# Autodesk Inventor assembly: ENSAMBLE GENERAL ACH-40L-2020-V
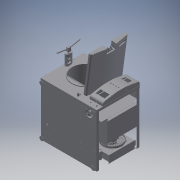
[picture p0: Inventor's stored thumbnail of the model, 180x180]
Saved by Autodesk Inventor 2017 (Build 210142000, 142)
## iProperties
Created: 2020-09-24
Part Number: ENSAMBLE GENERAL ACH-40L-2020-V
Description: STEP AP203
Document SubType Name: Assembly
Designer: USUARIO
Sending System: SolidWorks 2013
Preprocessor: SwSTEP 2.0
Title: ENSAMBLE GENERAL ACH-40L-2020-V.STEP
Revision Number: ANY
## Documents named in this file (46)
- D:\Laboratorio\Autoclave\Autoclave Horizontal\Sin Precamara\2020\Autoclave 40L con Vacio Insulab #0045883XX OP2020292\Ensamble General\ENSAMBLE GENERAL ACH-40L-2020-V.iam
- D:\Laboratorio\Autoclave\Autoclave Horizontal\Sin Precamara\2020\Autoclave 40L con Vacio Insulab #0045883XX OP2020292\Ensamble General\CUBIERTA FRONTAL ACH-40L-2020-V.ipt
- D:\Laboratorio\Autoclave\Autoclave Horizontal\Sin Precamara\2020\Autoclave 40L con Vacio Insulab #0045883XX OP2020292\Ensamble General\BASE MUEBLE ACH-40L-2020-V.ipt
- D:\Laboratorio\Autoclave\Autoclave Horizontal\Sin Precamara\2020\Autoclave 40L con Vacio Insulab #0045883XX OP2020292\Ensamble General\MARCO POSTERIOR ACH-40L-2020-V.ipt
- D:\Laboratorio\Autoclave\Autoclave Horizontal\Sin Precamara\2020\Autoclave 40L con Vacio Insulab #0045883XX OP2020292\Ensamble General\ENSAMBLE TANQUE ACH-40L-2020-V.iam
- D:\Laboratorio\Autoclave\Autoclave Horizontal\Sin Precamara\2020\Autoclave 40L con Vacio Insulab #0045883XX OP2020292\Ensamble General\ENSAMBLE PANEL FRONTAL ACH-40L-2020-V.iam
- D:\Laboratorio\Autoclave\Autoclave Horizontal\Sin Precamara\2020\Autoclave 40L con Vacio Insulab #0045883XX OP2020292\Ensamble General\ENSAMBLE PUERTA ACH-40L-2020-V.iam
- D:\Laboratorio\Autoclave\Autoclave Horizontal\Sin Precamara\2020\Autoclave 40L con Vacio Insulab #0045883XX OP2020292\Ensamble General\CAJA CONEXIONES ESPINAS ACH-40L-2020-V.ipt
- D:\Laboratorio\Autoclave\Autoclave Horizontal\Sin Precamara\2020\Autoclave 40L con Vacio Insulab #0045883XX OP2020292\Ensamble General\PG-13,5.ipt
- D:\Laboratorio\Autoclave\Autoclave Horizontal\Sin Precamara\2020\Autoclave 40L con Vacio Insulab #0045883XX OP2020292\Ensamble General\CAJA CONEXIONES ACH-40L-2020-V.ipt
- D:\Laboratorio\Autoclave\Autoclave Horizontal\Sin Precamara\2020\Autoclave 40L con Vacio Insulab #0045883XX OP2020292\Ensamble General\REFUERZO INTERIOR ACH-40L-2020-V.ipt
- D:\Laboratorio\Autoclave\Autoclave Horizontal\Sin Precamara\2020\Autoclave 40L con Vacio Insulab #0045883XX OP2020292\Ensamble General\VENTILADOR 9X9.ipt
- D:\Laboratorio\Autoclave\Autoclave Horizontal\Sin Precamara\2020\Autoclave 40L con Vacio Insulab #0045883XX OP2020292\Ensamble General\ENSAMBLE GENERAL CIERRE JP2019-TTNR.iam
- D:\Laboratorio\Autoclave\Autoclave Horizontal\Sin Precamara\2020\Autoclave 40L con Vacio Insulab #0045883XX OP2020292\Ensamble General\PIN CIERRE JP2019-TTNR.ipt
- D:\Laboratorio\Autoclave\Autoclave Horizontal\Sin Precamara\2020\Autoclave 40L con Vacio Insulab #0045883XX OP2020292\Ensamble General\PIN BISAGRA JP2019-TTNR.ipt
- D:\Laboratorio\Autoclave\Autoclave Horizontal\Sin Precamara\2020\Autoclave 40L con Vacio Insulab #0045883XX OP2020292\Ensamble General\PIVOTE CIERRE JP2019-TTNR.ipt
- D:\Laboratorio\Autoclave\Autoclave Horizontal\Sin Precamara\2020\Autoclave 40L con Vacio Insulab #0045883XX OP2020292\Ensamble General\ENSAMBLE TAPA ACH-40L-2020-V.iam
- D:\Laboratorio\Autoclave\Autoclave Horizontal\Sin Precamara\2020\Autoclave 40L con Vacio Insulab #0045883XX OP2020292\Ensamble General\ENSAMBLE RESERVORIO ACH-40L-2020-V.iam
- D:\Laboratorio\Autoclave\Autoclave Horizontal\Sin Precamara\2020\Autoclave 40L con Vacio Insulab #0045883XX OP2020292\Ensamble General\CONTRATAPA SUPERIOR ACH-40L-2020-V.ipt
- D:\Laboratorio\Autoclave\Autoclave Horizontal\Sin Precamara\2020\Autoclave 40L con Vacio Insulab #0045883XX OP2020292\Ensamble General\BANDEJA INTERIOR ACH-40L-2020-V.ipt
- D:\Laboratorio\Autoclave\Autoclave Horizontal\Sin Precamara\2020\Autoclave 40L con Vacio Insulab #0045883XX OP2020292\Ensamble General\BOMBA DE VACIO THOMAS 2107CA20.ipt
- D:\Laboratorio\Autoclave\Autoclave Horizontal\Sin Precamara\2020\Autoclave 40L con Vacio Insulab #0045883XX OP2020292\Ensamble General\CALDERIN ACH-40L-2020-V.ipt
- D:\Laboratorio\Autoclave\Autoclave Horizontal\Sin Precamara\2020\Autoclave 40L con Vacio Insulab #0045883XX OP2020292\Ensamble General\CONTRATAPA INFERIOR ACH-40L-2020-V.ipt
- D:\Laboratorio\Autoclave\Autoclave Horizontal\Sin Precamara\2020\Autoclave 40L con Vacio Insulab #0045883XX OP2020292\Ensamble General\CUBIERTA SUPERIOR ACH-40L-2020-V.ipt
- D:\Laboratorio\Autoclave\Autoclave Horizontal\Sin Precamara\2020\Autoclave 40L con Vacio Insulab #0045883XX OP2020292\Ensamble General\CUBIERTA LATERAL ACH-40L-2020-V.ipt
- D:\Laboratorio\Autoclave\Autoclave Horizontal\Sin Precamara\2020\Autoclave 40L con Vacio Insulab #0045883XX OP2020292\Ensamble General\ENSAMBLE RADIADOR ACH-40L-2020-V.iam
- D:\Laboratorio\Autoclave\Autoclave Horizontal\Sin Precamara\2020\Autoclave 40L con Vacio Insulab #0045883XX OP2020292\Ensamble General\CUBIERTA LATERAL DERECHA ACH-40L-2020-V.ipt
- D:\Laboratorio\Autoclave\Autoclave Horizontal\Sin Precamara\2020\Autoclave 40L con Vacio Insulab #0045883XX OP2020292\Ensamble General\CUBIERTA POSTERIOR ACH-40L-2020-V.ipt
- D:\Laboratorio\Autoclave\Autoclave Horizontal\Sin Precamara\2020\Autoclave 40L con Vacio Insulab #0045883XX OP2020292\Ensamble General\ULKA EX5.ipt
- D:\Laboratorio\Autoclave\Autoclave Horizontal\Sin Precamara\2020\Autoclave 40L con Vacio Insulab #0045883XX OP2020292\Ensamble General\DANFOSS EV215B.ipt
- D:\Laboratorio\Autoclave\Autoclave Horizontal\Sin Precamara\2020\Autoclave 40L con Vacio Insulab #0045883XX OP2020292\Ensamble General\SOPORTE BOMBA AGUA ACH-40L-2020-V.ipt
- D:\Laboratorio\Autoclave\Autoclave Horizontal\Sin Precamara\2020\Autoclave 40L con Vacio Insulab #0045883XX OP2020292\Ensamble General\SOPORTE VALVULAS ACH-40L-2020-V.ipt
- D:\Laboratorio\Autoclave\Autoclave Horizontal\Sin Precamara\2020\Autoclave 40L con Vacio Insulab #0045883XX OP2020292\Ensamble General\PATA 5-16.ipt
- D:\Laboratorio\Autoclave\Autoclave Horizontal\Sin Precamara\2020\Autoclave 40L con Vacio Insulab #0045883XX OP2020292\Ensamble General\VALVULA DE BOLA GENEBRE MH 3097-02 CW617N.ipt
- D:\Laboratorio\Autoclave\Autoclave Horizontal\Sin Precamara\2020\Autoclave 40L con Vacio Insulab #0045883XX OP2020292\Ensamble General\ESPINAS DE PESCADO ACV-ACH.ipt
- D:\Laboratorio\Autoclave\Autoclave Horizontal\Sin Precamara\2020\Autoclave 40L con Vacio Insulab #0045883XX OP2020292\Ensamble General\DERIVACION TANQUE ACH-40L-2020-V.ipt
- D:\Laboratorio\Autoclave\Autoclave Horizontal\Sin Precamara\2020\Autoclave 40L con Vacio Insulab #0045883XX OP2020292\Ensamble General\TEE VALVULAS ACH-40L-2020-V.ipt
- D:\Laboratorio\Autoclave\Autoclave Horizontal\Sin Precamara\2020\Autoclave 40L con Vacio Insulab #0045883XX OP2020292\Ensamble General\RESISTENCIA INTERIOR ACH-40L-2020-V.ipt
- D:\Laboratorio\Autoclave\Autoclave Horizontal\Sin Precamara\2020\Autoclave 40L con Vacio Insulab #0045883XX OP2020292\Ensamble General\RESISTENCIA SECADO ACH-40L-2020-V.ipt
- D:\Laboratorio\Autoclave\Autoclave Horizontal\Sin Precamara\2020\Autoclave 40L con Vacio Insulab #0045883XX OP2020292\Ensamble General\DEFLECTOR ACH-40L-2020-V.ipt
- D:\Laboratorio\Autoclave\Autoclave Horizontal\Sin Precamara\2020\Autoclave 40L con Vacio Insulab #0045883XX OP2020292\Ensamble General\ACOPLE DEFLECTOR ACH-40L-2020-V.ipt
- C:\Modelos 3D y DXF\Racores\B69 1-4x1-4.iam
- C:\Modelos 3D y DXF\Racores\B122 1-4x1-2.ipt
- C:\Modelos 3D y DXF\Racores\B116 1-4x1-4.ipt
- C:\Modelos 3D y DXF\Filtro en Y\Filtro Y 1-2'' Inox.ipt
- C:\Modelos 3D y DXF\Racores\Tuerca1.4.ipt
## Components (70 placed, 56 different names)
1. CUBIERTA FRONTAL ACH-40L-2020-V_1
2. BASE MUEBLE ACH-40L-2020-V_2 — Angle:2, Angle:3, Angle:4, Angle:5, Angle:6, Angle:7, Angle:8
3. MARCO POSTERIOR ACH-40L-2020-V_3
4. ENSAMBLE TANQUE ACH-40L-2020-V_4 [sub-assembly] — Insert:12
5. ENSAMBLE PANEL FRONTAL ACH-40L-2020-V_5 [sub-assembly]
6. ENSAMBLE PUERTA ACH-40L-2020-V_6 [sub-assembly]
7. CAJA CONEXIONES ESPINAS ACH-40L-2020-V_7
8. PG-13,5_8
9. CAJA CONEXIONES ACH-40L-2020-V_9
10. REFUERZO INTERIOR ACH-40L-2020-V_10
11. REFUERZO INTERIOR ACH-40L-2020-V_11
12. VENTILADOR 9X9_12
13. ENSAMBLE GENERAL CIERRE JP2019-TTNR_13 [sub-assembly]
14. PIN CIERRE JP2019-TTNR_14
15. PIN BISAGRA JP2019-TTNR_15
16. PIN BISAGRA JP2019-TTNR_16
17. PIVOTE CIERRE JP2019-TTNR_17
18. ENSAMBLE TAPA ACH-40L-2020-V_18 [sub-assembly]
19. ENSAMBLE RESERVORIO ACH-40L-2020-V_19 [sub-assembly]
20. CONTRATAPA SUPERIOR ACH-40L-2020-V_20
21. BANDEJA INTERIOR ACH-40L-2020-V_21
22. BOMBA DE VACIO THOMAS 2107CA20_22
23. CALDERIN ACH-40L-2020-V_23 — Insert:1, Angle:1
24. CONTRATAPA INFERIOR ACH-40L-2020-V_24
25. CUBIERTA SUPERIOR ACH-40L-2020-V_25
26. CUBIERTA LATERAL ACH-40L-2020-V_26
27. ENSAMBLE RADIADOR ACH-40L-2020-V_27 [sub-assembly]
28. CUBIERTA LATERAL DERECHA ACH-40L-2020-V_28
29. CUBIERTA POSTERIOR ACH-40L-2020-V_29
30. ULKA EX5_30
31. DANFOSS EV215B_31 — Insert:5, Insert:6
32. SOPORTE BOMBA AGUA ACH-40L-2020-V_32
33. SOPORTE VALVULAS ACH-40L-2020-V_33
34. DANFOSS EV215B_34 — Insert:17
35. DANFOSS EV215B_35 — Insert:15
36. DANFOSS EV215B_36 — Insert:7, Insert:14
37. DANFOSS EV215B_37 — Insert:18
38. DANFOSS EV215B_38 — Insert:16
39. PATA 5-16_39
40. PATA 5-16_40
41. PATA 5-16_41
42. PATA 5-16_42
43. PG-13,5_43
44. VALVULA DE BOLA GENEBRE MH 3097-02 CW617N_44
45. ESPINAS DE PESCADO ACV-ACH_45
46. DERIVACION TANQUE ACH-40L-2020-V_46 — Insert:8, Insert:9, Insert:10, Insert:11
47. TEE VALVULAS ACH-40L-2020-V_47
48. RESISTENCIA INTERIOR ACH-40L-2020-V_48
49. RESISTENCIA SECADO ACH-40L-2020-V_49
50. DEFLECTOR ACH-40L-2020-V_50
51. ACOPLE DEFLECTOR ACH-40L-2020-V_51
52. B116 1-4x1-4:1 — Insert:1, Angle:1, Insert:2
53. B122 1-4x1-2:1 — Insert:2, Insert:3
54. Filtro Y 1-2'' Inox:1 — Insert:3, Insert:4
55. B122 1-4x1-2:2 — Insert:4, Mate:1
56. Tuerca1.4:1 — Mate:1
57. B116 1-4x1-4:2 — Insert:5, Angle:2
58. B69 1-4x1-4:1 [sub-assembly] — Insert:6
59. B69 1-4x1-4:2 [sub-assembly] — Insert:7
60. B69 1-4x1-4:3 [sub-assembly] — Insert:8
61. B69 1-4x1-4:4 [sub-assembly] — Insert:9
62. B69 1-4x1-4:5 [sub-assembly] — Insert:10
63. B69 1-4x1-4:6 [sub-assembly] — Insert:11
64. B116 1-4x1-4:3 — Insert:12, Angle:3, Insert:13
65. B69 1-4x1-4:7 [sub-assembly] — Insert:13
66. B116 1-4x1-4:4 — Insert:16, Angle:6
67. B116 1-4x1-4:5 — Insert:14, Angle:4
68. B116 1-4x1-4:6 — Insert:15, Angle:5
69. B116 1-4x1-4:7 — Insert:17, Angle:7
70. B116 1-4x1-4:8 — Insert:18, Angle:8
## Relationships (27: Insert 18, Angle 8, Mate 1)
- Insert:1 (-7 mm): CALDERIN ACH-40L-2020-V_23 ↔ B116 1-4x1-4:1
- Angle:1 (0 deg): CALDERIN ACH-40L-2020-V_23 ↔ B116 1-4x1-4:1
- Insert:2 (-7 mm): B116 1-4x1-4:1 ↔ B122 1-4x1-2:1
- Insert:3 (7 mm): B122 1-4x1-2:1 ↔ Filtro Y 1-2'' Inox:1
- Insert:4 (-9 mm): Filtro Y 1-2'' Inox:1 ↔ B122 1-4x1-2:2
- Mate:1: B122 1-4x1-2:2 ↔ Tuerca1.4:1
- Insert:5 (-5 mm): DANFOSS EV215B_31 ↔ B116 1-4x1-4:2
- Angle:2 (179.9087 deg): BASE MUEBLE ACH-40L-2020-V_2 ↔ B116 1-4x1-4:2
- Insert:6 (-5 mm): DANFOSS EV215B_31 ↔ B69 1-4x1-4:1
- Insert:7 (7 mm): DANFOSS EV215B_36 ↔ B69 1-4x1-4:2
- Insert:8 (-5 mm): DERIVACION TANQUE ACH-40L-2020-V_46 ↔ B69 1-4x1-4:3
- Insert:9 (-5 mm): DERIVACION TANQUE ACH-40L-2020-V_46 ↔ B69 1-4x1-4:4
- Insert:10 (-5 mm): DERIVACION TANQUE ACH-40L-2020-V_46 ↔ B69 1-4x1-4:5
- Insert:11 (-5 mm): DERIVACION TANQUE ACH-40L-2020-V_46 ↔ B69 1-4x1-4:6
- Insert:12 (-7 mm): ENSAMBLE TANQUE ACH-40L-2020-V_4 ↔ B116 1-4x1-4:3
- Angle:3 (-91.6732 deg): BASE MUEBLE ACH-40L-2020-V_2 ↔ B116 1-4x1-4:3
- Insert:13 (-7 mm): B116 1-4x1-4:3 ↔ B69 1-4x1-4:7
- Insert:14 (-5 mm): DANFOSS EV215B_36 ↔ B116 1-4x1-4:5
- Insert:15 (10 mm): DANFOSS EV215B_35 ↔ B116 1-4x1-4:6
- Insert:16 (-5 mm): DANFOSS EV215B_38 ↔ B116 1-4x1-4:4
- Angle:4 (179.9087 deg): BASE MUEBLE ACH-40L-2020-V_2 ↔ B116 1-4x1-4:5
- Angle:5 (179.9087 deg): BASE MUEBLE ACH-40L-2020-V_2 ↔ B116 1-4x1-4:6
- Angle:6 (0 deg): BASE MUEBLE ACH-40L-2020-V_2 ↔ B116 1-4x1-4:4
- Insert:17 (-5 mm): DANFOSS EV215B_34 ↔ B116 1-4x1-4:7
- Insert:18 (-5 mm): DANFOSS EV215B_37 ↔ B116 1-4x1-4:8
- Angle:7 (91.6732 deg): BASE MUEBLE ACH-40L-2020-V_2 ↔ B116 1-4x1-4:7
- Angle:8 (-91.6732 deg): BASE MUEBLE ACH-40L-2020-V_2 ↔ B116 1-4x1-4:8
